# Autodesk Inventor assembly: rear_bumper
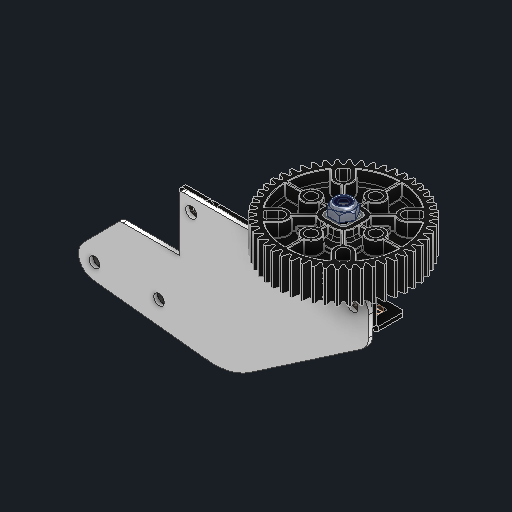
[picture p0: Inventor's stored thumbnail of the model, 512x512]
Saved by Autodesk Inventor 2024 (Build 280153000, 153)
## iProperties
Created: 2024-02-11
Part Number: rear_bumper
Document SubType Name: Assembly
Designer: Averey Ku
Author: Averey Ku
## Documents named in this file (15)
- D:\vex_robotics\hardware\cad\vroomba_v0.1\chassis\drivebay\rear_bumper.iam
- D:\vex_robotics\hardware\cad\vroomba_v0.1\custom_parts\drivebay\sled.ipt
- D:\vex_robotics\hardware\cad\VEX-CAD-Inventor-1.41\Structure\Angle\Aluminum 1x1\Alu Angle 1x1x6.ipt
- D:\vex_robotics\hardware\cad\VEX-CAD-Inventor-1.41\Motion\Spacers\Spacer Nylon .500 OD\NSpacer Black .500 OD x .375.ipt
- D:\vex_robotics\hardware\cad\VEX-CAD-Inventor-1.41\Motion\Spacers\Spacer Nylon .500 OD.ipt
- D:\vex_robotics\hardware\cad\VEX-CAD-Inventor-1.41\Motion\Spacers\Washer Steel\SWasher .375 OD x .062500.ipt
- D:\vex_robotics\hardware\cad\VEX-CAD-Inventor-1.41\Motion\Spacers\Washer Steel.ipt
- D:\vex_robotics\hardware\cad\VEX-CAD-Inventor-1.41\Motion\Spacers\Washer Teflon\TWasher .375 OD x .04000.ipt
- D:\vex_robotics\hardware\cad\VEX-CAD-Inventor-1.41\Motion\Spacers\Washer Teflon.ipt
- D:\vex_robotics\hardware\cad\VEX-CAD-Inventor-1.41\Structure\Hardware\Nut Keps.ipt
- D:\vex_robotics\hardware\cad\VEX-CAD-Inventor-1.41\Motion\Spacers\Spacer Nylon .375 OD\NSpacer .375 OD x .375.ipt
- D:\vex_robotics\hardware\cad\VEX-CAD-Inventor-1.41\Motion\Spacers\Spacer Nylon .375 OD.ipt
- D:\vex_robotics\hardware\cad\VEX-CAD-Inventor-1.41\Motion\Gears\HS Gear\HS 48T Gear, No Insert.iam
- D:\vex_robotics\hardware\cad\VEX-CAD-Inventor-1.41\Motion\Gears\HS Gear.iam
- D:\vex_robotics\hardware\cad\VEX-CAD-Inventor-1.41\Structure\Hardware\Nut Thin Nylock.ipt
## Components (14 placed, 9 different names)
1. sled:1 — Insert:1, Mate:1, Insert:8, Insert:9
2. Alu Angle 1x1x6:1 — Insert:1, Mate:1, Insert:2, Insert:3, Insert:13
3. NSpacer Black .500 OD x .375:1 — Insert:2
4. NSpacer Black .500 OD x .375:2 — Insert:3
5. SWasher .375 OD x .062500:1 — Insert:9
6. TWasher .375 OD x .04000:1
7. TWasher .375 OD x .04000:2
8. SWasher .375 OD x .062500:2 — Insert:8
9. TWasher .375 OD x .04000:3
10. TWasher .375 OD x .04000:4
11. Nut Keps:1 — Insert:13
12. NSpacer .375 OD x .375:1
13. HS 48T Gear, No Insert:1 [sub-assembly]
14. Nut Thin Nylock:1
## Relationships (14: Insert 13, Mate 1)
- Insert:1: sled:1 ↔ Alu Angle 1x1x6:1
- Mate:1: sled:1 ↔ Alu Angle 1x1x6:1
- Insert:2: Alu Angle 1x1x6:1 ↔ NSpacer Black .500 OD x .375:1
- Insert:3: Alu Angle 1x1x6:1 ↔ NSpacer Black .500 OD x .375:2
- [Insert]: TWasher .375 OD x .04000:1 ↔ TWasher .375 OD x .04000:2
- [Insert]: SWasher .375 OD x .062500:1 ↔ TWasher .375 OD x .04000:2
- [Insert]: TWasher .375 OD x .04000:3 ↔ TWasher .375 OD x .04000:4
- [Insert]: SWasher .375 OD x .062500:2 ↔ TWasher .375 OD x .04000:4
- Insert:8: sled:1 ↔ SWasher .375 OD x .062500:2
- Insert:9: sled:1 ↔ SWasher .375 OD x .062500:1
- [Insert]: Nut Keps:1 ↔ NSpacer .375 OD x .375:1
- [Insert]: NSpacer .375 OD x .375:1 ↔ HS 48T Gear, No Insert:1
- [Insert]: HS 48T Gear, No Insert:1 ↔ Nut Thin Nylock:1
- Insert:13: Alu Angle 1x1x6:1 ↔ Nut Keps:1
## Named parameters: d6_d22 = 0 mm, d7_d23 = 0 mm
